# Autodesk Inventor assembly: robot
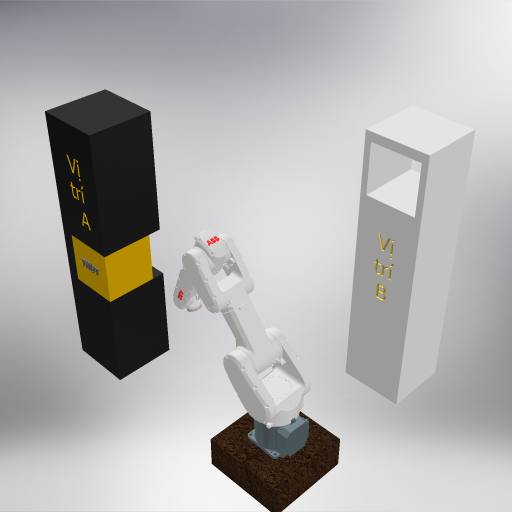
[picture p0: Inventor's stored thumbnail of the model, 512x512]
Saved by Autodesk Inventor 2023.3 (Build 273359000, 359)
## iProperties
Created: 2023-05-23
Part Number: robot
Document SubType Name: Assembly
Designer: Nguyen Xuan Lam
Author: Nguyen Xuan Lam
## Documents named in this file (10)
- C:\Users\Admin\Downloads\IRB 1300-1150_OmniCore_rev02_SAT_j\IRB 1300-1150_OmniCore_rev02_SAT_j\robot.iam
- C:\Users\Admin\Downloads\IRB 1300-1150_OmniCore_rev02_SAT_j\IRB 1300-1150_OmniCore_rev02_SAT_j\link0-bottom cable\link0-bottom cable.ipt
- C:\Users\Admin\Downloads\IRB 1300-1150_OmniCore_rev02_SAT_j\IRB 1300-1150_OmniCore_rev02_SAT_j\link1_1400\link1_1400.ipt
- C:\Users\Admin\Downloads\IRB 1300-1150_OmniCore_rev02_SAT_j\IRB 1300-1150_OmniCore_rev02_SAT_j\link2_1150\link2_1150.ipt
- C:\Users\Admin\Downloads\IRB 1300-1150_OmniCore_rev02_SAT_j\IRB 1300-1150_OmniCore_rev02_SAT_j\space.ipt
- C:\Users\Admin\Downloads\IRB 1300-1150_OmniCore_rev02_SAT_j\IRB 1300-1150_OmniCore_rev02_SAT_j\link4_900\link4_900.ipt
- C:\Users\Admin\Downloads\IRB 1300-1150_OmniCore_rev02_SAT_j\IRB 1300-1150_OmniCore_rev02_SAT_j\link3\link3.ipt
- C:\Users\Admin\Downloads\IRB 1300-1150_OmniCore_rev02_SAT_j\IRB 1300-1150_OmniCore_rev02_SAT_j\link5-foundry\link5-foundry.ipt
- C:\Users\Admin\Downloads\IRB 1300-1150_OmniCore_rev02_SAT_j\IRB 1300-1150_OmniCore_rev02_SAT_j\link6-foundry\link6-foundry.ipt
- C:\Users\Admin\Downloads\IRB 1300-1150_OmniCore_rev02_SAT_j\IRB 1300-1150_OmniCore_rev02_SAT_j\Part36.ipt
## Components (9 placed, 9 different names)
1. space:1 — Mate:3, Mate:4, Mate:16, Flush:1, Flush:2
2. link0-bottom cable:1 — Mate:1, Mate:2, Angle:1, Mate:3, Mate:4
3. link1_1400:1 — Mate:1, Mate:2, Angle:1, Mate:6, Mate:17
4. link2_1150:1 — Mate:6, Mate:7, Mate:9, Mate:17
5. link3:1 — Mate:7, Mate:9, Mate:10, Mate:11
6. link4_900:1 — Mate:10, Mate:11, Mate:12, Mate:13
7. link5-foundry:1 — Mate:12, Mate:13, Mate:14, Mate:15
8. link6-foundry:3 — Mate:14, Mate:15
9. Part36:1 — Mate:16, Flush:1, Flush:2
## Relationships (18: Mate 15, Flush 2, Angle 1)
- Mate:1 (-31.81 mm): link0-bottom cable:1 ↔ link1_1400:1
- Mate:2 (2.317 mm): link0-bottom cable:1 ↔ link1_1400:1
- Angle:1 (0 deg): link0-bottom cable:1 ↔ link1_1400:1
- Mate:3: space:1 ↔ link0-bottom cable:1
- Mate:4: space:1 ↔ link0-bottom cable:1
- Mate:6: link1_1400:1 ↔ link2_1150:1
- Mate:7: link2_1150:1 ↔ link3:1
- Mate:9: link2_1150:1 ↔ link3:1
- Mate:10: link3:1 ↔ link4_900:1
- Mate:11: link3:1 ↔ link4_900:1
- Mate:12: link4_900:1 ↔ link5-foundry:1
- Mate:13: link4_900:1 ↔ link5-foundry:1
- Mate:14: link5-foundry:1 ↔ link6-foundry:3
- Mate:15: link5-foundry:1 ↔ link6-foundry:3
- Mate:16: space:1 ↔ Part36:1
- Flush:1: space:1 ↔ Part36:1
- Flush:2: space:1 ↔ Part36:1
- Mate:17: link1_1400:1 ↔ link2_1150:1
